# Autodesk Inventor assembly: RoArm_ensamble
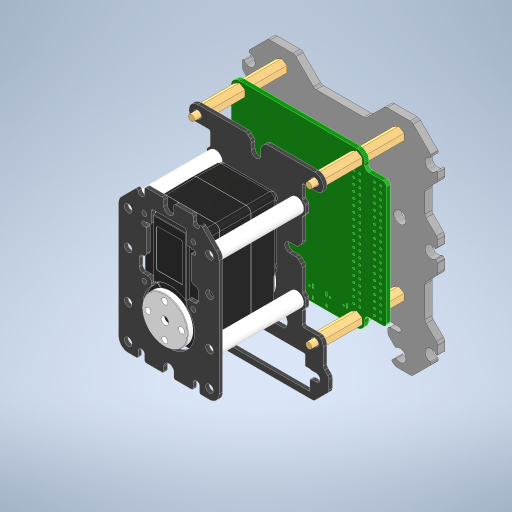
[picture p0: Inventor's stored thumbnail of the model, 512x512]
Saved by Autodesk Inventor 2024.4 (Build 284460000, 460)
## iProperties
Created: 2026-06-02
Part Number: RoArm_ensamble
Document SubType Name: Assembly
Designer: epm01
Author: epm01
## Documents named in this file (8)
- D:\Archivos\2026-2\RoArm\inventor\RoArm_ensamble.iam
- D:\Archivos\2026-2\RoArm\inventor\Base\Base\Base.ipt
- D:\Archivos\2026-2\RoArm\inventor\Poste_inf\Poste_inf\Poste_inf.ipt
- D:\Archivos\2026-2\RoArm\inventor\Board\Board\Board.ipt
- D:\Archivos\2026-2\RoArm\inventor\base_sup\base_sup\base_sup.ipt
- D:\Archivos\2026-2\RoArm\inventor\poste_nylon\poste_nylon\poste_nylon.ipt
- D:\Archivos\2026-2\RoArm\inventor\ST3215 v1\ST3215 v1\ST3215 v1.iam
- D:\Archivos\2026-2\RoArm\inventor\base_sup_motor\base_sup_motor\base_sup_motor.ipt
## Components (17 placed, 7 different names)
1. Base:1 — Mate:1, Mate:2, Mate:3, Mate:4
2. Poste_inf:1 — Mate:7
3. Poste_inf:2 — Mate:2
4. Poste_inf:3 — Mate:3
5. Poste_inf:4 — Mate:4
6. Poste_inf:5 — Mate:9, Mate:10
7. Poste_inf:6 — Mate:6
8. Poste_inf:7 — Mate:1, Mate:5
9. Poste_inf:8 — Mate:8
10. Board:1 — Mate:5, Mate:6, Mate:7, Mate:8, Mate:9
11. base_sup:1 — Mate:10, Insert:1, Insert:2, Insert:3, Insert:4, Flush:1
12. poste_nylon:1 — Insert:2
13. poste_nylon:2 — Insert:1
14. poste_nylon:3 — Insert:4
15. poste_nylon:4 — Insert:3, Insert:5
16. ST3215 v1:1 [sub-assembly] — Insert:6, Flush:2
17. base_sup_motor:1 — Insert:5, Flush:1, Insert:6, Flush:2
## Relationships (18: Mate 10, Insert 6, Flush 2)
- Mate:1: Base:1 ↔ Poste_inf:7
- Mate:2: Base:1 ↔ Poste_inf:2
- Mate:3: Base:1 ↔ Poste_inf:3
- Mate:4: Base:1 ↔ Poste_inf:4
- Mate:5: Poste_inf:7 ↔ Board:1
- Mate:6: Poste_inf:6 ↔ Board:1
- Mate:7: Poste_inf:1 ↔ Board:1
- Mate:8: Poste_inf:8 ↔ Board:1
- Mate:9: Poste_inf:5 ↔ Board:1
- Mate:10: Poste_inf:5 ↔ base_sup:1
- Insert:1: base_sup:1 ↔ poste_nylon:2
- Insert:2: base_sup:1 ↔ poste_nylon:1
- Insert:3: base_sup:1 ↔ poste_nylon:4
- Insert:4: base_sup:1 ↔ poste_nylon:3
- Insert:5: poste_nylon:4 ↔ base_sup_motor:1
- Flush:1: base_sup:1 ↔ base_sup_motor:1
- Insert:6: ST3215 v1:1 ↔ base_sup_motor:1
- Flush:2: ST3215 v1:1 ↔ base_sup_motor:1
